# Autodesk Inventor assembly: Foot
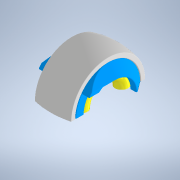
[picture p0: Inventor's stored thumbnail of the model, 180x180]
Saved by Autodesk Inventor 2022.2 (Build 262287030, 287C)
## iProperties
Created: 2021-12-28
Part Number: Foot
Document SubType Name: Assembly
Designer: Jochen
Author: Jochen
## Documents named in this file (4)
- D:\Projects\Lisbeth\CAD\foot\Foot.iam
- D:\Projects\Lisbeth\CAD\foot\Toe.ipt
- D:\Projects\Lisbeth\CAD\foot\ToePalm.ipt
- D:\Projects\Lisbeth\CAD\Foot\ToeDampenerStressed.ipt
## Components (4 placed, 3 different names)
1. Toe:1 — Mate:7, Mate:8, Mate:9
2. ToePalm:1 — Mate:7, Mate:8, Mate:9
3. ToeDampenerStressed:1 — Mate:11, Mate:12
4. ToeDampenerStressed:2 — Mate:10, Mate:13
## Relationships (7: Mate 7)
- Mate:7: Toe:1 ↔ ToePalm:1
- Mate:8: Toe:1 ↔ ToePalm:1
- Mate:9: Toe:1 ↔ ToePalm:1
- Mate:10: ToeDampenerStressed:2
- Mate:11: ToeDampenerStressed:1
- Mate:12 (-5.25 mm): ToeDampenerStressed:1
- Mate:13 (-5.25 mm): ToeDampenerStressed:2
